# Autodesk Inventor assembly: Montagem1
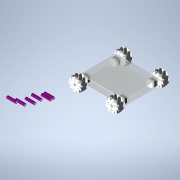
[picture p0: Inventor's stored thumbnail of the model, 180x180]
Saved by Autodesk Inventor 2021 (Build 250183000, 183)
## iProperties
Created: 2022-03-22
Part Number: Montagem1
Document SubType Name: Assembly
Designer: aluno
Author: aluno
## Documents named in this file (5)
- U:\Projeto\Montagem1.iam
- U:\Projeto\Base.ipt
- U:\Projeto\Mecanum.iam
- U:\Projeto\MINEBEA 05701607 stepper motor.ipt
- U:\Projeto\INR18650-35E Samsung.ipt
## Components (16 placed, 4 different names)
1. Base:2 — Coincidente:5, Coincidente:6, Alinhado:13, Coincidente:7, Alinhado:14, Alinhado:15, Coincidente:8, Alinhado:16, Alinhado:17, Coincidente:9, Alinhado:18, Alinhado:19, Coincidente:20, Coincidente:21
2. Mecanum:5 [sub-assembly] — Coincidente:10, Coincidente:13
3. Mecanum:6 [sub-assembly] — Coincidente:14, Coincidente:15
4. Mecanum:7 [sub-assembly] — Coincidente:12, Coincidente:17
5. Mecanum:8 [sub-assembly] — Coincidente:11, Coincidente:16
6. MINEBEA 05701607 stepper motor:5 — Coincidente:9, Alinhado:18, Alinhado:19, Coincidente:14, Coincidente:15, Coincidente:18, Alinhado:20, Alinhado:21
7. MINEBEA 05701607 stepper motor:6 — Coincidente:5, Coincidente:6, Alinhado:13, Coincidente:11, Coincidente:16
8. MINEBEA 05701607 stepper motor:7 — Coincidente:8, Alinhado:16, Alinhado:17, Coincidente:12, Coincidente:17
9. INR18650-35E Samsung:1
10. INR18650-35E Samsung:2
11. INR18650-35E Samsung:3 — Tangente:1, Alinhado:22
12. INR18650-35E Samsung:4
13. INR18650-35E Samsung:5 — Tangente:1, Alinhado:22
14. INR18650-35E Samsung:6
15. MINEBEA 05701607 stepper motor:8 — Coincidente:7, Alinhado:14, Alinhado:15, Coincidente:10, Coincidente:13, Coincidente:19
16. Base:3 — Coincidente:18, Alinhado:20, Alinhado:21, Coincidente:19, Coincidente:20, Coincidente:21
## Relationships (28: Mate 17, Flush 10, Tangent 1)
- Coincidente:5 [Mate]: Base:2 ↔ MINEBEA 05701607 stepper motor:6
- Coincidente:6 [Mate]: Base:2 ↔ MINEBEA 05701607 stepper motor:6
- Alinhado:13 [Flush] (3 mm): Base:2 ↔ MINEBEA 05701607 stepper motor:6
- Coincidente:7 [Mate]: Base:2 ↔ MINEBEA 05701607 stepper motor:8
- Alinhado:14 [Flush] (3 mm): Base:2 ↔ MINEBEA 05701607 stepper motor:8
- Alinhado:15 [Flush]: Base:2 ↔ MINEBEA 05701607 stepper motor:8
- Coincidente:8 [Mate]: Base:2 ↔ MINEBEA 05701607 stepper motor:7
- Alinhado:16 [Flush]: Base:2 ↔ MINEBEA 05701607 stepper motor:7
- Alinhado:17 [Flush] (3 mm): Base:2 ↔ MINEBEA 05701607 stepper motor:7
- Coincidente:9 [Mate]: Base:2 ↔ MINEBEA 05701607 stepper motor:5
- Alinhado:18 [Flush]: Base:2 ↔ MINEBEA 05701607 stepper motor:5
- Alinhado:19 [Flush] (3 mm): Base:2 ↔ MINEBEA 05701607 stepper motor:5
- Coincidente:10 [Mate]: Mecanum:5 ↔ MINEBEA 05701607 stepper motor:8
- Coincidente:11 [Mate]: Mecanum:8 ↔ MINEBEA 05701607 stepper motor:6
- Coincidente:12 [Mate]: Mecanum:7 ↔ MINEBEA 05701607 stepper motor:7
- Coincidente:13 [Mate] (10 mm): Mecanum:5 ↔ MINEBEA 05701607 stepper motor:8
- Coincidente:14 [Mate]: Mecanum:6 ↔ MINEBEA 05701607 stepper motor:5
- Coincidente:15 [Mate] (10 mm): Mecanum:6 ↔ MINEBEA 05701607 stepper motor:5
- Coincidente:16 [Mate] (10 mm): Mecanum:8 ↔ MINEBEA 05701607 stepper motor:6
- Coincidente:17 [Mate] (10 mm): Mecanum:7 ↔ MINEBEA 05701607 stepper motor:7
- Coincidente:18 [Mate]: MINEBEA 05701607 stepper motor:5 ↔ Base:3
- Alinhado:20 [Flush]: MINEBEA 05701607 stepper motor:5 ↔ Base:3
- Alinhado:21 [Flush]: MINEBEA 05701607 stepper motor:5 ↔ Base:3
- Coincidente:19 [Mate]: MINEBEA 05701607 stepper motor:8 ↔ Base:3
- Coincidente:20 [Mate]: Base:2 ↔ Base:3
- Coincidente:21 [Mate]: Base:2 ↔ Base:3
- Tangente:1: INR18650-35E Samsung:3 ↔ INR18650-35E Samsung:5
- Alinhado:22 [Flush]: INR18650-35E Samsung:3 ↔ INR18650-35E Samsung:5
